# Autodesk Inventor assembly: Slope_testasm
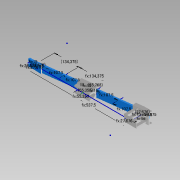
[picture p0: Inventor's stored thumbnail of the model, 180x180]
Saved by Autodesk Inventor 2021 (Build 250183000, 183)
## iProperties
Created: 2021-03-11
Part Number: Slope_testasm
Document SubType Name: Assembly
Designer: kumagai
Author: kumagai
## Documents named in this file (7)
- X:\Develop\CAD\PlaRails\SimpleSlope\Slope_testasm.iam
- X:\Develop\CAD\PlaRails\SimpleSlope\Slope_LowEnd_C.ipt
- X:\Develop\CAD\PlaRails\SimpleSlope\Slope_Middle_C.ipt
- X:\Develop\CAD\PlaRails\StraightRail\StraightRail_i\StraightMF215.iam
- X:\Develop\CAD\PlaRails\StraightRail\StraightRail_i.iam
- X:\Develop\CAD\PlaRails\SimpleSlope\SlopeProfile.ipt
- X:\Develop\CAD\PlaRails\SimpleSlope\Slope_HighEnd_C.ipt
## Components (6 placed, 5 different names)
1. Slope_LowEnd_C:1 — フラッシュ:1, フラッシュ:2, メイト:2, フラッシュ:3, メイト:3, フラッシュ:5
2. Slope_Middle_C:1 — フラッシュ:1, フラッシュ:2, メイト:1, フラッシュ:4, メイト:4, フラッシュ:6, メイト:6
3. StraightMF215:1 [sub-assembly] — メイト:1, メイト:2, フラッシュ:3, メイト:3
4. SlopeProfile:1
5. Slope_HighEnd_C:1 — フラッシュ:4, フラッシュ:5, メイト:5
6. StraightMF215:2 [sub-assembly] — メイト:4, メイト:5, フラッシュ:6, メイト:6
## Relationships (12: Flush 6, Mate 6)
- フラッシュ:1 [Flush]: Slope_LowEnd_C:1 ↔ Slope_Middle_C:1
- フラッシュ:2 [Flush]: Slope_LowEnd_C:1 ↔ Slope_Middle_C:1
- メイト:1 [Mate]: Slope_Middle_C:1 ↔ StraightMF215:1
- メイト:2 [Mate]: Slope_LowEnd_C:1 ↔ StraightMF215:1
- フラッシュ:3 [Flush]: Slope_LowEnd_C:1 ↔ StraightMF215:1
- メイト:3 [Mate]: Slope_LowEnd_C:1 ↔ StraightMF215:1
- フラッシュ:4 [Flush]: Slope_Middle_C:1 ↔ Slope_HighEnd_C:1
- フラッシュ:5 [Flush]: Slope_LowEnd_C:1 ↔ Slope_HighEnd_C:1
- メイト:4 [Mate]: Slope_Middle_C:1 ↔ StraightMF215:2
- メイト:5 [Mate]: Slope_HighEnd_C:1 ↔ StraightMF215:2
- フラッシュ:6 [Flush]: Slope_Middle_C:1 ↔ StraightMF215:2
- メイト:6 [Mate]: Slope_Middle_C:1 ↔ StraightMF215:2
